# Autodesk Inventor assembly: Assembled
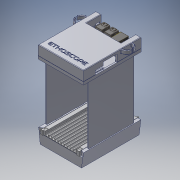
[picture p0: Inventor's stored thumbnail of the model, 180x180]
Saved by Autodesk Inventor 2017 (Build 210142000, 142)
## iProperties
Created: 2017-05-28
Part Number: Assembled
Document SubType Name: Assembly
Designer: Paolo
Author: Paolo
## Documents named in this file (13)
- E:\Rymapt_projects\Ethoscope\ethoscope_hardware\Assembled.iam
- E:\Rymapt_projects\Ethoscope\ethoscope_hardware\core\lower_pi_case\lowerPiCase.ipt
- E:\Rymapt_projects\Ethoscope\ethoscope_hardware\core\light_box\core_lightBox.ipt
- E:\Rymapt_projects\Ethoscope\ethoscope_hardware\core\RPi3\RasPi_Camera.ipt
- E:\Rymapt_projects\Ethoscope\ethoscope_hardware\core\RPi3\RPi3_ModelB.ipt
- E:\Rymapt_projects\Ethoscope\ethoscope_hardware\core\side_wall\SideWall_new.ipt
- E:\Rymapt_projects\Ethoscope\ethoscope_hardware\core\side_wall\LIghtTile_new.ipt
- E:\Rymapt_projects\Ethoscope\ethoscope_hardware\core\upper_pi_case\upperPiCase_new.ipt
- E:\Rymapt_projects\Ethoscope\ethoscope_hardware\arenas\arena_10x1_longTubes\arena_10x1_longTubes.ipt
- C:\Users\Paolo\Documents\Disegni\CAD\MyParts\2017_05_Screw_M2\pan_head_phillip_mc_screw_m2.ipt
- C:\Users\Paolo\Documents\Disegni\CAD\MyParts\2017_05_Screw_M2\Hex Nut\M2.ipt
- C:\Users\Paolo\Documents\Disegni\CAD\MyParts\2017_05_Screw_M2\M3\M3 x 0.5mm Thread 12mm LONG SOCKET HEAD CAP SCREW.ipt
- C:\Users\Paolo\Documents\Disegni\CAD\MyParts\2017_05_Screw_M2\M3\M3 x 0.5mm Thread HEX NUT.ipt
## Components (21 placed, 12 different names)
1. upperPiCase_new:1 — Mate:6, Mate:7, Flush:1
2. RasPi_Camera:1 — Mate:1, Mate:2, Angle:1, Mate:20, Mate:21
3. RPi3_ModelB:1 — Mate:3, Mate:4, Angle:2, Mate:25, Mate:26
4. lowerPiCase:1 — Mate:1, Mate:2, Angle:1, Mate:3, Mate:4, Angle:2, Mate:6, Mate:7, Flush:1, Flush:3, Flush:4, Mate:10, Flush:5, Flush:6, Mate:12, Insert:2, Insert:3, Mate:22, Mate:23, Mate:28, Mate:29, Mate:30, Mate:31, Mate:32, Mate:33, Mate:34, Mate:35, Mate:36, Mate:37
5. SideWall_new:2 — Flush:4, Mate:10, Mate:11, Flush:5, Flush:7, Mate:14
6. SideWall_new:3 — Flush:6, Mate:12, Mate:13, Flush:7
7. core_lightBox:1 — Flush:3, Mate:11, Mate:13, Flush:8, Mate:14, Mate:15, Mate:16, Mate:17
8. LIghtTile_new:1 — Flush:8
9. arena_10x1_longTubes:1 — Mate:15, Mate:16, Mate:17
10. pan_head_phillip_mc_screw_m2:1 — Insert:3, Mate:19
11. pan_head_phillip_mc_screw_m2:2 — Insert:2, Mate:18
12. M2:1 — Mate:19, Mate:21
13. M2:2 — Mate:18, Mate:20
14. M3 x 0.5mm Thread 12mm LONG SOCKET HEAD CAP SCREW:3 — Mate:30, Mate:31
15. M3 x 0.5mm Thread 12mm LONG SOCKET HEAD CAP SCREW:4 — Mate:32, Mate:33
16. M3 x 0.5mm Thread 12mm LONG SOCKET HEAD CAP SCREW:5 — Mate:35, Mate:36
17. M3 x 0.5mm Thread 12mm LONG SOCKET HEAD CAP SCREW:6 — Mate:34, Mate:37
18. M3 x 0.5mm Thread 12mm LONG SOCKET HEAD CAP SCREW:1 — Mate:22, Mate:27, Mate:28
19. M3 x 0.5mm Thread HEX NUT:2 — Mate:26, Mate:27
20. M3 x 0.5mm Thread 12mm LONG SOCKET HEAD CAP SCREW:2 — Mate:23, Mate:24, Mate:29
21. M3 x 0.5mm Thread HEX NUT:1 — Mate:24, Mate:25
## Relationships (45: Mate 34, Flush 7, Angle 2, Insert 2)
- Mate:1: RasPi_Camera:1 ↔ lowerPiCase:1
- Mate:2: RasPi_Camera:1 ↔ lowerPiCase:1
- Angle:1 (0 deg): RasPi_Camera:1 ↔ lowerPiCase:1
- Mate:3: RPi3_ModelB:1 ↔ lowerPiCase:1
- Mate:4: RPi3_ModelB:1 ↔ lowerPiCase:1
- Angle:2 (0 deg): RPi3_ModelB:1 ↔ lowerPiCase:1
- Mate:6: upperPiCase_new:1 ↔ lowerPiCase:1
- Mate:7 (0.5 mm): upperPiCase_new:1 ↔ lowerPiCase:1
- Flush:1: upperPiCase_new:1 ↔ lowerPiCase:1
- Flush:3: lowerPiCase:1 ↔ core_lightBox:1
- Flush:4 (1.8 mm): lowerPiCase:1 ↔ SideWall_new:2
- Mate:10 (0.2 mm): lowerPiCase:1 ↔ SideWall_new:2
- Mate:11 (0.2 mm): SideWall_new:2 ↔ core_lightBox:1
- Flush:5 (-13 mm): lowerPiCase:1 ↔ SideWall_new:2
- Flush:6 (1.8 mm): lowerPiCase:1 ↔ SideWall_new:3
- Mate:12 (0.2 mm): lowerPiCase:1 ↔ SideWall_new:3
- Mate:13 (0.2 mm): SideWall_new:3 ↔ core_lightBox:1
- Flush:7: SideWall_new:2 ↔ SideWall_new:3
- Flush:8: core_lightBox:1 ↔ LIghtTile_new:1
- Mate:14 (1.3 mm): SideWall_new:2 ↔ core_lightBox:1
- Mate:15: core_lightBox:1 ↔ arena_10x1_longTubes:1
- Mate:16: core_lightBox:1 ↔ arena_10x1_longTubes:1
- Mate:17: core_lightBox:1 ↔ arena_10x1_longTubes:1
- Insert:2 (-7.95 mm): lowerPiCase:1 ↔ pan_head_phillip_mc_screw_m2:2
- Insert:3 (-7.95 mm): lowerPiCase:1 ↔ pan_head_phillip_mc_screw_m2:1
- Mate:18: pan_head_phillip_mc_screw_m2:2 ↔ M2:2
- Mate:19: pan_head_phillip_mc_screw_m2:1 ↔ M2:1
- Mate:20 (0.2 mm): RasPi_Camera:1 ↔ M2:2
- Mate:21 (0.2 mm): RasPi_Camera:1 ↔ M2:1
- Mate:22: lowerPiCase:1 ↔ M3 x 0.5mm Thread 12mm LONG SOCKET HEAD CAP SCREW:1
- Mate:23: lowerPiCase:1 ↔ M3 x 0.5mm Thread 12mm LONG SOCKET HEAD CAP SCREW:2
- Mate:24: M3 x 0.5mm Thread 12mm LONG SOCKET HEAD CAP SCREW:2 ↔ M3 x 0.5mm Thread HEX NUT:1
- Mate:25 (0.2 mm): RPi3_ModelB:1 ↔ M3 x 0.5mm Thread HEX NUT:1
- Mate:26 (0.2 mm): RPi3_ModelB:1 ↔ M3 x 0.5mm Thread HEX NUT:2
- Mate:27: M3 x 0.5mm Thread 12mm LONG SOCKET HEAD CAP SCREW:1 ↔ M3 x 0.5mm Thread HEX NUT:2
- Mate:28 (0.2 mm): lowerPiCase:1 ↔ M3 x 0.5mm Thread 12mm LONG SOCKET HEAD CAP SCREW:1
- Mate:29 (0.2 mm): lowerPiCase:1 ↔ M3 x 0.5mm Thread 12mm LONG SOCKET HEAD CAP SCREW:2
- Mate:30: lowerPiCase:1 ↔ M3 x 0.5mm Thread 12mm LONG SOCKET HEAD CAP SCREW:3
- Mate:31 (0.2 mm): lowerPiCase:1 ↔ M3 x 0.5mm Thread 12mm LONG SOCKET HEAD CAP SCREW:3
- Mate:32: lowerPiCase:1 ↔ M3 x 0.5mm Thread 12mm LONG SOCKET HEAD CAP SCREW:4
- Mate:33 (0.2 mm): lowerPiCase:1 ↔ M3 x 0.5mm Thread 12mm LONG SOCKET HEAD CAP SCREW:4
- Mate:34: lowerPiCase:1 ↔ M3 x 0.5mm Thread 12mm LONG SOCKET HEAD CAP SCREW:6
- Mate:35: lowerPiCase:1 ↔ M3 x 0.5mm Thread 12mm LONG SOCKET HEAD CAP SCREW:5
- Mate:36 (0.2 mm): lowerPiCase:1 ↔ M3 x 0.5mm Thread 12mm LONG SOCKET HEAD CAP SCREW:5
- Mate:37 (0.2 mm): lowerPiCase:1 ↔ M3 x 0.5mm Thread 12mm LONG SOCKET HEAD CAP SCREW:6
